# Autodesk Inventor assembly: CableBraider
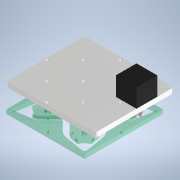
[picture p0: Inventor's stored thumbnail of the model, 180x180]
Saved by Autodesk Inventor 2020.2 (Build 242310000, 310)
## iProperties
Created: 2020-07-21
Part Number: CableBraider
Document SubType Name: Assembly
Designer: elmar
Author: elmar
## Documents named in this file (6)
- D:\FourWireBraidingMachine\InventorFiles\CableBraider.iam
- D:\FourWireBraidingMachine\InventorFiles\BasePlate.ipt
- D:\FourWireBraidingMachine\InventorFiles\DriveGear.ipt
- D:\FourWireBraidingMachine\InventorFiles\NEMA17.ipt
- D:\FourWireBraidingMachine\InventorFiles\HornGear.ipt
- D:\FourWireBraidingMachine\InventorFiles\GuidePlate.ipt
## Components (5 placed, 5 different names)
1. BasePlate:1 — Mate:1, Mate:2, Mate:3, Insert:1, Angle:1, Insert:2, Insert:3, Angle:2, Insert:4
2. DriveGear:1 — Insert:2
3. BraiderMotor — Insert:1, Angle:1
4. HornGear:1 — Insert:3
5. GuidePlate:1 — Angle:2, Insert:4
## Relationships (9: Insert 4, Mate 3, Angle 2)
- Mate:1: BasePlate:1
- Mate:2: BasePlate:1
- Mate:3: BasePlate:1
- Insert:1: BasePlate:1 ↔ BraiderMotor
- Angle:1 (0 deg): BasePlate:1 ↔ BraiderMotor
- Insert:2: BasePlate:1 ↔ DriveGear:1
- Insert:3: BasePlate:1 ↔ HornGear:1
- Angle:2 (0 deg): BasePlate:1 ↔ GuidePlate:1
- Insert:4 (40 mm): BasePlate:1 ↔ GuidePlate:1
